# Autodesk Inventor assembly: highlander
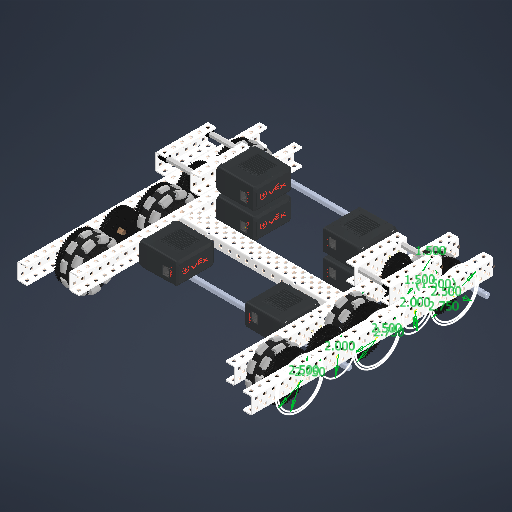
[picture p0: Inventor's stored thumbnail of the model, 512x512]
Saved by Autodesk Inventor 2025.1 (Build 291241000, 241)
## iProperties
Created: 2025-07-20
Part Number: highlander
Document SubType Name: Assembly
Designer: Exortions
Author: Exortions
## Documents named in this file (16)
- D:\Robotics\jank-2025-3284B\cad3284b-2025\highlander\highlander.iam
- D:\Robotics\jank-2025-3284B\cad3284b-2025\VEX-CAD-Inventor-1.4.2\Structure\C Channel\Aluminum 1x2x1\Alu C 1x2x1x28.ipt
- D:\Robotics\jank-2025-3284B\cad3284b-2025\VEX-CAD-Inventor-1.4.2\Structure\C Channel\Aluminum 1x2x1\Alu C 1x2x1x26.ipt
- D:\Robotics\jank-2025-3284B\cad3284b-2025\highlander\parts\hs-drivetrain-crossbrace.iam
- D:\Robotics\jank-2025-3284B\cad3284b-2025\VEX-CAD-Inventor-1.4.2\Structure\C Channel\Aluminum 1x2x1\Alu C 1x2x1x6.ipt
- D:\Robotics\jank-2025-3284B\cad3284b-2025\VEX-CAD-Inventor-1.4.2\Structure\C Channel\Aluminum 1x2x1\Alu C 1x2x1x19.ipt
- D:\Robotics\jank-2025-3284B\cad3284b-2025\VEX-CAD-Inventor-1.4.2\Electronics\V5 Motor.ipt
- D:\Robotics\jank-2025-3284B\cad3284b-2025\VEX-CAD-Inventor-1.4.2\Motion\Spacers\Spacer Nylon .375 OD\NSpacer .375 OD x .375.ipt
- D:\Robotics\jank-2025-3284B\cad3284b-2025\VEX-CAD-Inventor-1.4.2\Motion\Spacers\Spacer Nylon .375 OD.ipt
- D:\Robotics\jank-2025-3284B\cad3284b-2025\VEX-CAD-Inventor-1.4.2\Motion\Spacers\Washer Teflon\TWasher .375 OD x .06250.ipt
- D:\Robotics\jank-2025-3284B\cad3284b-2025\VEX-CAD-Inventor-1.4.2\Motion\Spacers\Washer Teflon.ipt
- D:\Robotics\jank-2025-3284B\cad3284b-2025\VEX-CAD-Inventor-1.4.2\Structure\Standoff\Standoff 1.50.ipt
- D:\Robotics\jank-2025-3284B\cad3284b-2025\VEX-CAD-Inventor-1.4.2\Structure\Standoff.ipt
- D:\Robotics\jank-2025-3284B\cad3284b-2025\highlander\parts\drivetrain-wheel.iam
- D:\Robotics\jank-2025-3284B\cad3284b-2025\highlander\parts\halfcut-48t-gear.iam
- D:\Robotics\jank-2025-3284B\cad3284b-2025\VEX-CAD-Inventor-1.4.2\Motion\Gears\LS 36T Gear.ipt
## Components (42 placed, 12 different names)
1. Alu C 1x2x1x28:1 — Insert:3, Insert:4, Mate:19, Insert:8, Mate:20, Insert:37, Insert:38, Insert:39, Insert:40, Insert:41
2. Alu C 1x2x1x26:2 — Mate:15, Insert:6, Mate:17, Mate:18, Insert:10, Mate:22, Insert:23, Mate:25, Insert:24, Mate:26
3. Alu C 1x2x1x28:2 — Mate:16, Insert:7, Mate:17, Insert:11, Mate:23, Insert:44, Insert:45, Insert:46, Insert:48, Insert:49
4. Alu C 1x2x1x26:3 — Mate:14, Insert:5, Mate:18, Mate:19, Insert:9, Mate:21, Insert:14, Insert:15, Insert:16, Insert:17, Insert:18, Insert:19
5. hs-drivetrain-crossbrace:2 [sub-assembly] — Insert:3, Mate:14, Mate:15, Mate:16
6. hs-drivetrain-crossbrace:3 [sub-assembly] — Insert:4, Insert:5, Insert:6, Insert:7
7. Alu C 1x2x1x6:1 — Insert:8, Mate:20, Insert:27, Insert:34, Insert:43
8. Alu C 1x2x1x6:2 — Insert:9, Mate:21, Insert:20, Insert:21
9. Alu C 1x2x1x6:3 — Insert:10, Mate:22, Insert:22, Mate:24
10. Alu C 1x2x1x6:4 — Insert:11, Mate:23, Insert:35, Insert:36
11. V5 Motor:1 — Insert:20, Insert:21
12. V5 Motor:2 — Insert:14, Insert:15
13. V5 Motor:3 — Insert:23, Mate:25
14. V5 Motor:4 — Insert:22, Mate:24
15. V5 Motor:5 — Insert:16, Insert:17
16. Alu C 1x2x1x19:1 — Insert:18, Insert:19
17. V5 Motor:6 — Insert:24, Mate:26
18. NSpacer .375 OD x .375:1 — Insert:25, Insert:26
19. TWasher .375 OD x .06250:1 — Insert:26, Insert:27
20. Standoff 1.50:1 — Insert:25
21. NSpacer .375 OD x .375:2
22. TWasher .375 OD x .06250:2 — Insert:34
23. Standoff 1.50:2
24. NSpacer .375 OD x .375:3
25. TWasher .375 OD x .06250:3 — Insert:36
26. Standoff 1.50:3
27. NSpacer .375 OD x .375:4
28. TWasher .375 OD x .06250:4 — Insert:35
29. Standoff 1.50:4
30. drivetrain-wheel:1 [sub-assembly] — Insert:37
31. drivetrain-wheel:2 [sub-assembly] — Insert:38
32. drivetrain-wheel:3 [sub-assembly] — Insert:39
33. halfcut-48t-gear:1 [sub-assembly] — Insert:40
34. halfcut-48t-gear:2 [sub-assembly] — Insert:41, Insert:42
35. LS 36T Gear:1 — Insert:42
36. LS 36T Gear:2 — Insert:43
37. drivetrain-wheel:4 [sub-assembly] — Insert:44
38. drivetrain-wheel:5 [sub-assembly] — Insert:45
39. drivetrain-wheel:6 [sub-assembly] — Insert:46
40. halfcut-48t-gear:3 [sub-assembly] — Insert:48
41. halfcut-48t-gear:4 [sub-assembly] — Insert:49
42. LS 36T Gear:3
## Relationships (58: Insert 45, Mate 13)
- Insert:3 (9.525 mm): Alu C 1x2x1x28:1 ↔ hs-drivetrain-crossbrace:2
- Mate:14: Alu C 1x2x1x26:3 ↔ hs-drivetrain-crossbrace:2
- Mate:15: Alu C 1x2x1x26:2 ↔ hs-drivetrain-crossbrace:2
- Mate:16: Alu C 1x2x1x28:2 ↔ hs-drivetrain-crossbrace:2
- Insert:4 (19.05 mm): Alu C 1x2x1x28:1 ↔ hs-drivetrain-crossbrace:3
- Insert:5 (19.05 mm): Alu C 1x2x1x26:3 ↔ hs-drivetrain-crossbrace:3
- Insert:6 (19.05 mm): Alu C 1x2x1x26:2 ↔ hs-drivetrain-crossbrace:3
- Insert:7 (19.05 mm): Alu C 1x2x1x28:2 ↔ hs-drivetrain-crossbrace:3
- Mate:17: Alu C 1x2x1x26:2 ↔ Alu C 1x2x1x28:2
- Mate:18: Alu C 1x2x1x26:2 ↔ Alu C 1x2x1x26:3
- Mate:19: Alu C 1x2x1x28:1 ↔ Alu C 1x2x1x26:3
- Insert:8 (12.7 mm): Alu C 1x2x1x28:1 ↔ Alu C 1x2x1x6:1
- Mate:20: Alu C 1x2x1x28:1 ↔ Alu C 1x2x1x6:1
- Insert:9 (12.7 mm): Alu C 1x2x1x26:3 ↔ Alu C 1x2x1x6:2
- Mate:21: Alu C 1x2x1x26:3 ↔ Alu C 1x2x1x6:2
- Insert:10 (12.7 mm): Alu C 1x2x1x26:2 ↔ Alu C 1x2x1x6:3
- Mate:22: Alu C 1x2x1x26:2 ↔ Alu C 1x2x1x6:3
- Insert:11 (12.7 mm): Alu C 1x2x1x28:2 ↔ Alu C 1x2x1x6:4
- Mate:23: Alu C 1x2x1x28:2 ↔ Alu C 1x2x1x6:4
- Insert:14: Alu C 1x2x1x26:3 ↔ V5 Motor:2
- Insert:15: Alu C 1x2x1x26:3 ↔ V5 Motor:2
- Insert:16: Alu C 1x2x1x26:3 ↔ V5 Motor:5
- Insert:17: Alu C 1x2x1x26:3 ↔ V5 Motor:5
- Insert:18: Alu C 1x2x1x26:3 ↔ Alu C 1x2x1x19:1
- Insert:19: Alu C 1x2x1x26:3 ↔ Alu C 1x2x1x19:1
- Insert:20: Alu C 1x2x1x6:2 ↔ V5 Motor:1
- Insert:21: Alu C 1x2x1x6:2 ↔ V5 Motor:1
- Insert:22: Alu C 1x2x1x6:3 ↔ V5 Motor:4
- Mate:24: Alu C 1x2x1x6:3 ↔ V5 Motor:4
- Insert:23: Alu C 1x2x1x26:2 ↔ V5 Motor:3
- Mate:25: Alu C 1x2x1x26:2 ↔ V5 Motor:3
- Insert:24: Alu C 1x2x1x26:2 ↔ V5 Motor:6
- Mate:26: Alu C 1x2x1x26:2 ↔ V5 Motor:6
- Insert:25: NSpacer .375 OD x .375:1 ↔ Standoff 1.50:1
- Insert:26: NSpacer .375 OD x .375:1 ↔ TWasher .375 OD x .06250:1
- Insert:27: Alu C 1x2x1x6:1 ↔ TWasher .375 OD x .06250:1
- [Insert]: NSpacer .375 OD x .375:2 ↔ Standoff 1.50:2
- [Insert]: NSpacer .375 OD x .375:2 ↔ TWasher .375 OD x .06250:2
- [Insert]: NSpacer .375 OD x .375:3 ↔ Standoff 1.50:3
- [Insert]: NSpacer .375 OD x .375:3 ↔ TWasher .375 OD x .06250:3
- [Insert]: NSpacer .375 OD x .375:4 ↔ Standoff 1.50:4
- [Insert]: NSpacer .375 OD x .375:4 ↔ TWasher .375 OD x .06250:4
- Insert:34: Alu C 1x2x1x6:1 ↔ TWasher .375 OD x .06250:2
- Insert:35: Alu C 1x2x1x6:4 ↔ TWasher .375 OD x .06250:4
- Insert:36: Alu C 1x2x1x6:4 ↔ TWasher .375 OD x .06250:3
- Insert:37 (15.875 mm): Alu C 1x2x1x28:1 ↔ drivetrain-wheel:1
- Insert:38 (15.875 mm): Alu C 1x2x1x28:1 ↔ drivetrain-wheel:2
- Insert:39 (15.875 mm): Alu C 1x2x1x28:1 ↔ drivetrain-wheel:3
- Insert:40 (15.875 mm): Alu C 1x2x1x28:1 ↔ halfcut-48t-gear:1
- Insert:41 (15.875 mm): Alu C 1x2x1x28:1 ↔ halfcut-48t-gear:2
- Insert:42 (-6.35 mm): halfcut-48t-gear:2 ↔ LS 36T Gear:1
- Insert:43 (22.225 mm): Alu C 1x2x1x6:1 ↔ LS 36T Gear:2
- Insert:44 (15.875 mm): Alu C 1x2x1x28:2 ↔ drivetrain-wheel:4
- Insert:45 (15.875 mm): Alu C 1x2x1x28:2 ↔ drivetrain-wheel:5
- Insert:46 (15.875 mm): Alu C 1x2x1x28:2 ↔ drivetrain-wheel:6
- [Insert] (-6.35 mm): halfcut-48t-gear:4 ↔ LS 36T Gear:3
- Insert:48 (15.875 mm): Alu C 1x2x1x28:2 ↔ halfcut-48t-gear:3
- Insert:49 (15.875 mm): Alu C 1x2x1x28:2 ↔ halfcut-48t-gear:4
## Named parameters: d93_d90 = 0 mm, d94_d91 = 0 mm, d95_d90 = 0 mm, d96_d91 = 0 mm, d97_d90 = 0 mm, d98_d91 = 0 mm, d112_d107 = -6.35 mm
